# Autodesk Inventor assembly: CompleteRobotAssembly_NERDS
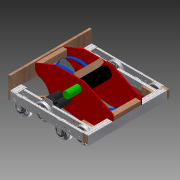
[picture p0: Inventor's stored thumbnail of the model, 180x180]
Saved by Autodesk Inventor 2014 (Build 180170000, 170)
## iProperties
Created: 2016-01-30
Part Number: CompleteRobotAssembly_NERDS
Document SubType Name: Assembly
Designer: bermudezr
Author: bermudezr
## Documents named in this file (5)
- C:\Users\choices.CTE\Documents\Nerds_1726\Models\2015-2016\Assemblies\Robot\Complete.iam
- C:\Users\choices.CTE\Documents\Nerds_1726\Models\2015-2016\Assemblies\Robot\Shooter.iam
- C:\Users\choices.CTE\Documents\Nerds_1726\Models\2015-2016\Assemblies\Robot\Chassis.iam
- C:\Users\choices.CTE\Documents\Nerds_1726\Models\2015-2016\Parts\Robot\Shooter\BallGuide.ipt
- C:\Users\choices.CTE\Documents\Nerds_1726\Models\2015-2016\Parts\Robot\Shooter\BallGuideLeft.ipt
## Components (4 placed, 4 different names)
1. Shooter:1 [sub-assembly] — Mate:4, Mate:5, Flush:2, Mate:6, Flush:3, Mate:10
2. Chassis:1 [sub-assembly] — Mate:4, Mate:5, Flush:2, Mate:6, Flush:3, Mate:7, Mate:8, Mate:9, Mate:11, Mate:12
3. BallGuide:1 — Mate:7, Mate:8, Mate:9
4. BallGuideLeft:1 — Mate:10, Mate:11, Mate:12
## Relationships (11: Mate 9, Flush 2)
- Mate:4: Shooter:1 ↔ Chassis:1
- Mate:5: Shooter:1 ↔ Chassis:1
- Flush:2: Shooter:1 ↔ Chassis:1
- Mate:6: Shooter:1 ↔ Chassis:1
- Flush:3: Shooter:1 ↔ Chassis:1
- Mate:7: Chassis:1 ↔ BallGuide:1
- Mate:8: Chassis:1 ↔ BallGuide:1
- Mate:9: Chassis:1 ↔ BallGuide:1
- Mate:10: Shooter:1 ↔ BallGuideLeft:1
- Mate:11: Chassis:1 ↔ BallGuideLeft:1
- Mate:12: Chassis:1 ↔ BallGuideLeft:1
